# Autodesk Inventor assembly: komplet_kol_V4
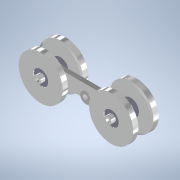
[picture p0: Inventor's stored thumbnail of the model, 180x180]
Saved by Autodesk Inventor 2020.3 (Build 243373000, 373)
## iProperties
Created: 2021-10-24
Part Number: komplet_kol_V4
Document SubType Name: Assembly
Designer: patry
Author: patry
## Documents named in this file (4)
- C:\Users\patry\Desktop\Konar staff\Ariadna2.1\ariadna_mechanika\Obszar roboczy\Naped\Zawieszenie_v3\komplet_kol_V4.iam
- C:\Users\patry\Desktop\Konar staff\Ariadna2.1\ariadna_mechanika\Obszar roboczy\Naped\Zawieszenie_v3\lacznik_pary_kol_V3.ipt
- C:\Users\patry\Desktop\Konar staff\Ariadna2.1\ariadna_mechanika\Obszar roboczy\Naped\Zawieszenie_v3\tuleja_TUF106040.ipt
- C:\Users\patry\Desktop\Konar staff\Ariadna2.1\ariadna_mechanika\Obszar roboczy\Naped\Kola\wheel_pair.iam
## Components (5 placed, 3 different names)
1. lacznik_pary_kol_V3:1
2. tuleja_TUF106040:1
3. tuleja_TUF106040:2
4. wheel_pair:1 [sub-assembly]
5. wheel_pair:2 [sub-assembly]
## Relationships (10: Mate 8, Angle 2)
- [Mate]: lacznik_pary_kol_V3:1 ↔ tuleja_TUF106040:1
- [Mate]: lacznik_pary_kol_V3:1 ↔ tuleja_TUF106040:1
- [Mate]: lacznik_pary_kol_V3:1 ↔ tuleja_TUF106040:2
- [Mate]: lacznik_pary_kol_V3:1 ↔ tuleja_TUF106040:2
- [Angle] (0 deg): lacznik_pary_kol_V3:1 ↔ tuleja_TUF106040:2
- [Angle] (0 deg): lacznik_pary_kol_V3:1 ↔ tuleja_TUF106040:1
- [Mate]: lacznik_pary_kol_V3:1 ↔ wheel_pair:1
- [Mate]: lacznik_pary_kol_V3:1 ↔ wheel_pair:1
- [Mate]: lacznik_pary_kol_V3:1 ↔ wheel_pair:2
- [Mate]: lacznik_pary_kol_V3:1 ↔ wheel_pair:2
